# Autodesk Inventor assembly: s-assy-guide
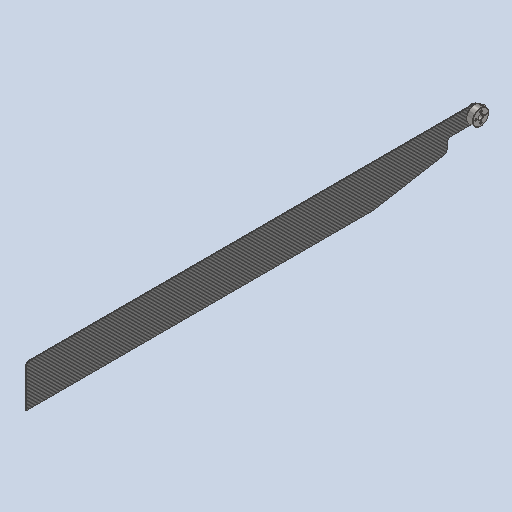
[picture p0: Inventor's stored thumbnail of the model, 512x512]
Saved by Autodesk Inventor 2022 (Build 260153000, 153)
## iProperties
Created: 2021-10-03
Part Number: s-assy-guide
Document SubType Name: Assembly
Designer: Yuta Kage
Author: Yuta Kage
## Documents named in this file (4)
- C:\Users\yuta0\Desktop\catchrobo_hardware-main\catchrobo_hardware-main\assy-shooter\s-assy-guide.iam
- C:\Users\yuta0\Desktop\catchrobo_hardware-main\catchrobo_hardware-main\assy-shooter\shooter_carbon_plate5.ipt
- C:\Users\yuta0\Desktop\catchrobo_hardware-main\catchrobo_hardware-main\assy-shooter\SCSTR6-8.iam
- C:\Users\yuta0\Desktop\catchrobo_hardware-main\catchrobo_hardware-main\assy-shooter\CB3-8.ipt
## Components (5 placed, 3 different names)
1. s_carbon_plate5:1 — メイト:1, メイト:2, メイト:3, メイト:4, メイト:5
2. SCSTR6-8:1 [sub-assembly] — メイト:1, メイト:2, メイト:3
3. CB3-8:1 — メイト:4, メイト:5
4. CB3-8:2
5. CB3-8:3
## Component patterns: (3 elements, first: CB3-8:1)
## Relationships (5: Mate 5)
- メイト:1 [Mate]: s_carbon_plate5:1 ↔ SCSTR6-8:1
- メイト:2 [Mate]: s_carbon_plate5:1 ↔ SCSTR6-8:1
- メイト:3 [Mate]: s_carbon_plate5:1 ↔ SCSTR6-8:1
- メイト:4 [Mate]: s_carbon_plate5:1 ↔ CB3-8:1
- メイト:5 [Mate]: s_carbon_plate5:1 ↔ CB3-8:1
